# Autodesk Inventor assembly: SidePanel_v2_left
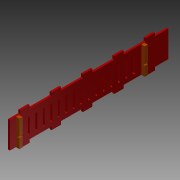
[picture p0: Inventor's stored thumbnail of the model, 180x180]
Saved by Autodesk Inventor 2015 SP1 (Build 190203100, 203)
## iProperties
Created: 2015-01-20
Part Number: SidePanel_v2_left
Document SubType Name: Assembly
Designer: Patrick
Author: Patrick
## Documents named in this file (3)
- C:\Users\Patrick\CAD\Spin5 Enclosure\SidePanel_v2_left.iam
- C:\Users\Patrick\CAD\Spin5 Enclosure\PCBSupport.ipt
- C:\Users\Patrick\CAD\Spin5 Enclosure\SidePanel_Rail_v2_vert.ipt
## Components (3 placed, 2 different names)
1. PCBSupport:1 — Rigid:1
2. PCBSupport:2 — Rigid:2
3. SidePanel_Rail_v2_vert:1 — Rigid:1, Rigid:2
## Relationships (2: WeldJoint 2)
- Rigid:1 [WeldJoint]: PCBSupport:1 ↔ SidePanel_Rail_v2_vert:1
- Rigid:2 [WeldJoint]: PCBSupport:2 ↔ SidePanel_Rail_v2_vert:1
